# Autodesk Inventor assembly: Link_Flame_16
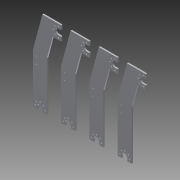
[picture p0: Inventor's stored thumbnail of the model, 180x180]
Saved by Autodesk Inventor 2013 (Build 170138000, 138)
## iProperties
Created: 2014-04-21
Part Number: Link_Flame_16
Document SubType Name: Assembly
Designer: andou
Author: andou
## Documents named in this file (2)
- C:\Users\andou\Documents\GitHub\Robotics-Project\design\RoboticsProject\project_4\cnc_data\Link_Flame_16.iam
- C:\Users\andou\Documents\GitHub\Robotics-Project\design\RoboticsProject\project_4\cnc_data\Leg_Link_Flame.ipt
## Components (4 placed, 1 different names)
1. Leg_Link_Flame:1
2. Leg_Link_Flame:2
3. Leg_Link_Flame:3
4. Leg_Link_Flame:4
## Component patterns: (4 elements, first: Leg_Link_Flame:1)
